# Autodesk Inventor assembly: power_distribution
Saved by Autodesk Inventor 2021 (Build 250183000, 183)
## iProperties
Created: 2021-01-22
Part Number: power_distribution
Document SubType Name: Assembly
Designer: User
Author: User
## Documents named in this file (5)
- D:\SynologyDrive\tcodev\tco-cad\common\power_distribution\power_distribution.iam
- D:\SynologyDrive\tcodev\tco-cad\common\power_distribution\Board.ipt
- D:\SynologyDrive\tcodev\tco-cad\common\kicad_packages_3d\PinHeader_1x02_P2.54mm_Vertical.ipt
- D:\SynologyDrive\tcodev\tco-cad\common\te_parts\usb_1903814_1.ipt
- D:\SynologyDrive\tcodev\tco-cad\common\kicad_packages_3d\PinHeader_1x05_P2.54mm_Vertical.ipt
## Components (6 placed, 4 different names)
1. Board:1 — Mate:1, Mate:2, Rigid:1, Rigid:2, Mate:5, Angle:1, Slider:1, Rigid:3, Rigid:4
2. PinHeader_1x02_P2.54mm_Vertical:1 — Mate:1, Rigid:1
3. PinHeader_1x02_P2.54mm_Vertical:2 — Mate:2, Rigid:2
4. PinHeader_1x05_P2.54mm_Vertical:1 — Rigid:4
5. PinHeader_1x05_P2.54mm_Vertical:2 — Rigid:3
6. usb_1903814_1:1 — Mate:5, Angle:1, Slider:1
## Relationships (11: Mate 5, WeldJoint 4, Angle 1, TranslationJoint 1)
- Mate:1: Board:1 ↔ PinHeader_1x02_P2.54mm_Vertical:1
- Mate:2: Board:1 ↔ PinHeader_1x02_P2.54mm_Vertical:2
- [Mate]: Board:1 ↔ PinHeader_1x05_P2.54mm_Vertical:1
- [Mate]: Board:1 ↔ PinHeader_1x05_P2.54mm_Vertical:2
- Rigid:1 [WeldJoint] (-3 mm): Board:1 ↔ PinHeader_1x02_P2.54mm_Vertical:1
- Rigid:2 [WeldJoint] (-3 mm): Board:1 ↔ PinHeader_1x02_P2.54mm_Vertical:2
- Mate:5: Board:1 ↔ usb_1903814_1:1
- Angle:1 (0 deg): Board:1 ↔ usb_1903814_1:1
- Slider:1 [TranslationJoint] (-2.84 mm): Board:1 ↔ usb_1903814_1:1
- Rigid:3 [WeldJoint] (-3 mm): Board:1 ↔ PinHeader_1x05_P2.54mm_Vertical:2
- Rigid:4 [WeldJoint] (-3 mm): Board:1 ↔ PinHeader_1x05_P2.54mm_Vertical:1
